# Autodesk Inventor assembly: Balancing Robot_10
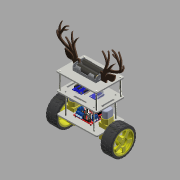
[picture p0: Inventor's stored thumbnail of the model, 180x180]
Saved by Autodesk Inventor 2019 (Build 230136000, 136)
## iProperties
Created: 2023-11-03
Part Number: Balancing Robot_10
Document SubType Name: Assembly
Designer: Vincent
Mass: 307.95 g
Surface Area: 1684.43 cm^2
Volume: 206.056 cm^3
Density: 1.49449 g/cm^3
Author: Vincent
## Documents named in this file (15)
- C:\Users\User\Downloads\Self Balancing Robot__7.iam
- C:\Users\User\Downloads\plate1.ipt
- C:\Users\User\Downloads\2 dc-motor-with-wheel-1.snapshot.3\dc_motor_with_wheel.ipt
- C:\Users\User\Downloads\2 dc-motor-with-wheel-1.snapshot.3\dc_motor_with_wheel_MIR.ipt
- C:\Users\User\Downloads\baut4.ipt
- C:\Users\User\Downloads\4 puente-h-l298-1.snapshot.1\Assembly1.iam
- C:\Users\User\Downloads\plate2.ipt
- C:\Users\User\Downloads\baut3.ipt
- C:\Users\User\Downloads\baut2.ipt
- C:\Users\User\Downloads\5 itg-mpu-gy-521-MPU6050-1.snapshot.16.zip (Unzipped Files)-20231029T034015Z-001\5 itg-mpu-gy-521-MPU6050-1.snapshot.16.zip (Unzipped Files)\ITG-MPU.ipt
- C:\Users\User\Downloads\3 wemos-d1-mini-v3-0-0-1.snapshot.1\WEMOS_D1_MINI_V3.0.0_MIR.ipt
- C:\Users\User\Downloads\plate3 - Copy.ipt
- C:\Users\User\Downloads\Battery Assembly.iam
- C:\Users\User\Downloads\deer2 - Copy.ipt
- C:\Users\User\Downloads\deer2 - Copy_MIR.ipt
## Components (23 placed, 14 different names)
1. plate1:1 — Mate:1, Mate:2, Insert:1, Insert:2, Insert:3, Insert:4, Insert:8, Insert:9, Insert:10, Insert:11
2. dc_motor_with_wheel:1 — Mate:1
3. dc_motor_with_wheel_MIR:1 — Mate:2
4. baut4:1 — Insert:1, Insert:6
5. baut4:2 — Insert:2
6. baut4:3 — Insert:3, Insert:5
7. baut4:4 — Insert:4
8. Assembly1:1 [sub-assembly] — Insert:5, Insert:6
9. plate2:1 — Insert:12, Insert:13, Mate:3, Mate:4, Insert:19, Insert:20
10. baut3:1 — Insert:15, Insert:19
11. baut3:2 — Insert:14
12. baut2:1 — Insert:8, Insert:13
13. baut2:2 — Insert:10
14. baut2:4 — Insert:9
15. baut2:5 — Insert:11, Insert:12
16. ITG-MPU:1 — Mate:4
17. WEMOS_D1_MINI_V3.0.0_MIR:1 — Mate:3
18. plate3 - Copy:1 — Insert:14, Insert:15, Insert:17, Insert:18, Mate:5, Mate:8, Mate:9
19. baut3:4 — Insert:17, Insert:20
20. baut3:5 — Insert:18
21. Battery Assembly:1 [sub-assembly] — Mate:5
22. deer2 - Copy:1 — Mate:8
23. deer2 - Copy_MIR:1 — Mate:9
## Relationships (25: Insert 18, Mate 7)
- Mate:1: plate1:1 ↔ dc_motor_with_wheel:1
- Mate:2: plate1:1 ↔ dc_motor_with_wheel_MIR:1
- Insert:1: plate1:1 ↔ baut4:1
- Insert:2: plate1:1 ↔ baut4:2
- Insert:3: plate1:1 ↔ baut4:3
- Insert:4: plate1:1 ↔ baut4:4
- Insert:5: baut4:3 ↔ Assembly1:1
- Insert:6: baut4:1 ↔ Assembly1:1
- Insert:8: plate1:1 ↔ baut2:1
- Insert:9: plate1:1 ↔ baut2:4
- Insert:10: plate1:1 ↔ baut2:2
- Insert:11: plate1:1 ↔ baut2:5
- Insert:12: plate2:1 ↔ baut2:5
- Insert:13: plate2:1 ↔ baut2:1
- Mate:3: plate2:1 ↔ WEMOS_D1_MINI_V3.0.0_MIR:1
- Mate:4: plate2:1 ↔ ITG-MPU:1
- Insert:14: baut3:2 ↔ plate3 - Copy:1
- Insert:15: baut3:1 ↔ plate3 - Copy:1
- Insert:17: plate3 - Copy:1 ↔ baut3:4
- Insert:18: plate3 - Copy:1 ↔ baut3:5
- Insert:19: plate2:1 ↔ baut3:1
- Insert:20: plate2:1 ↔ baut3:4
- Mate:5 (20 mm): plate3 - Copy:1 ↔ Battery Assembly:1
- Mate:8: plate3 - Copy:1 ↔ deer2 - Copy:1
- Mate:9: plate3 - Copy:1 ↔ deer2 - Copy_MIR:1
